# Autodesk Inventor assembly: Wheel
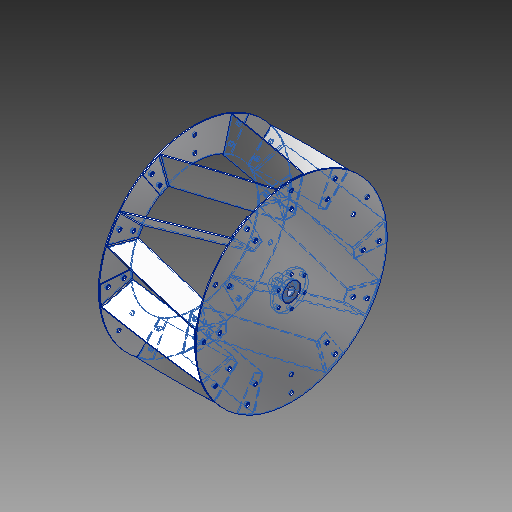
[picture p0: Inventor's stored thumbnail of the model, 512x512]
Saved by Autodesk Inventor 2019 (Build 230136000, 136)
## iProperties
Created: 2017-04-20
Part Number: Wheel
Document SubType Name: Assembly
Designer: Adhikara
Mass: 1032.4 g
Surface Area: 4830.7 cm^2
Volume: 382.369 cm^3
Density: 2.7 g/cm^3
Author: Adhikara
## Documents named in this file (5)
- C:\Users\Adhik\Documents\CAD\Julie\Wheel.iam
- C:\Users\Adhik\Documents\CAD\Julie\Wall.ipt
- C:\Users\Adhik\Documents\CAD\Julie\Edge.ipt
- C:\Users\Adhik\Documents\CAD\Julie\Rim.ipt
- C:\Users\Adhik\Documents\CAD\Julie\Key Hub.ipt
## Components (9 placed, 4 different names)
1. Wall:1 — Mate:1, Mate:2, Mate:3, Mate:4, Mate:5, Mate:6, Mate:10, Mate:11
2. Rim:1 — Mate:7, Mate:8
3. Key Hub:1 — Mate:9, Mate:10, Mate:11
4. Edge:2 — Mate:4, Mate:5, Mate:6, Mate:8
5. Edge:1 — Mate:1, Mate:2, Mate:3
6. Edge:3
7. Edge:4
8. Edge:5
9. Edge:6
## Component patterns: (3 elements, first: Edge:2 + Edge:1)
## Relationships (11: Mate 11)
- Mate:1: Wall:1 ↔ Edge:1
- Mate:2: Wall:1 ↔ Edge:1
- Mate:3: Wall:1 ↔ Edge:1
- Mate:4: Wall:1 ↔ Edge:2
- Mate:5: Wall:1 ↔ Edge:2
- Mate:6: Wall:1 ↔ Edge:2
- Mate:7: Rim:1
- Mate:8: Rim:1 ↔ Edge:2
- Mate:9: Key Hub:1
- Mate:10: Wall:1 ↔ Key Hub:1
- Mate:11: Wall:1 ↔ Key Hub:1
